# Autodesk Inventor assembly: Montagem para cotas
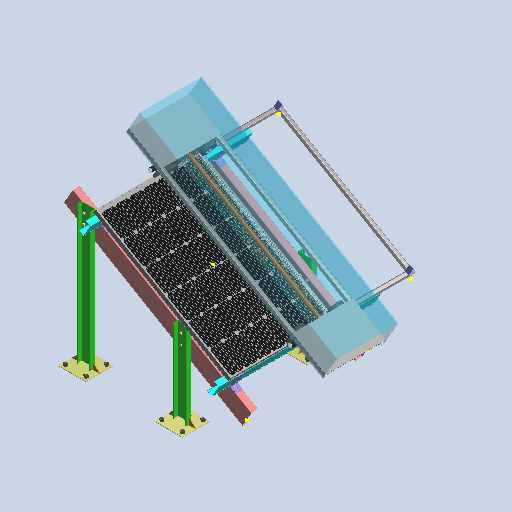
[picture p0: Inventor's stored thumbnail of the model, 512x512]
Saved by Autodesk Inventor 2026.2 (Build 302298010, 298A)
## iProperties
Created: 2019-12-15
Part Number: Montagem para cotas
Document SubType Name: Assembly
Designer: Rubens
Sending System: SolidWorks 2021
Last Author: Mohsen
Last Saved: 2022-08-25
Author: Rubens
## Documents named in this file (29)
- C:\Users\Rubens\Downloads\TCC1803\TCC 1703\Projeto TCC\Main_Solar_Structure\Montagem para cotas.iam
- C:\Users\Rubens\Downloads\TCC1803\TCC 1703\Projeto TCC\Main_Solar_Structure\Small_Column.ipt
- C:\Users\Rubens\Downloads\TCC1803\TCC 1703\Projeto TCC\Main_Solar_Structure\Large_Column.ipt
- C:\Users\Rubens\Downloads\TCC1803\TCC 1703\Projeto TCC\Main_Solar_Structure\Bottom_Beam.ipt
- C:\Users\Rubens\Downloads\TCC1803\TCC 1703\Projeto TCC\Main_Solar_Structure\Base_Plate.ipt
- C:\Users\Rubens\Downloads\TCC1803\TCC 1703\Projeto TCC\Main_Solar_Structure\Base_Support.ipt
- C:\Users\Rubens\Downloads\TCC1803\TCC 1703\Projeto TCC\Main_Solar_Structure\Beam_Support.ipt
- C:\Users\Rubens\Downloads\TCC1803\TCC 1703\Projeto TCC\Main_Solar_Structure\M10_Screw&Nut.iam
- C:\Users\Rubens\Downloads\TCC1803\TCC 1703\Projeto TCC\Main_Solar_Structure\ISO - 4034 - M16 - S_.ipt
- C:\Users\Rubens\Downloads\TCC1803\TCC 1703\Projeto TCC\Main_Solar_Structure\Base_Plate_MIR.ipt
- C:\Users\Rubens\Downloads\TCC1803\TCC 1703\Projeto TCC\Main_Solar_Structure\Base_Support_MIR.ipt
- C:\Users\Rubens\Downloads\TCC1803\TCC 1703\Projeto TCC\Main_Solar_Structure\ISO - 4034 - M16 - S__MIR.ipt
- C:\Users\Rubens\Downloads\TCC1803\TCC 1703\Projeto TCC\Main_Solar_Structure\Top_Beam_2780.ipt
- C:\Users\Rubens\Downloads\TCC1803\TCC 1703\Projeto TCC\Main_Solar_Structure\Perfil tubo - 30x30x3.ipt
- C:\Users\Rubens\Downloads\TCC1803\TCC 1703\Projeto TCC\Main_Solar_Structure\tubo 30 x 30 x 3  - 500.ipt
- C:\Users\Rubens\Downloads\TCC1803\TCC 1703\Projeto TCC\Main_Solar_Structure\Limitador.ipt
- C:\Users\Rubens\Downloads\TCC1803\TCC 1703\Projeto TCC\Projeto Limpador\MontagemREVXX.iam
- C:\Users\Rubens\Downloads\TCC1803\TCC 1703\Projeto TCC\Projeto Limpador\PV ST SOLAR.ipt
- C:\Users\Rubens\Downloads\TCC1803\TCC 1703\Projeto TCC\Main_Solar_Structure\Small_Column_MIR3.ipt
- C:\Users\Rubens\Downloads\TCC1803\TCC 1703\Projeto TCC\Main_Solar_Structure\Bottom_Beam_MIR3.ipt
- C:\Users\Rubens\Downloads\TCC1803\TCC 1703\Projeto TCC\Main_Solar_Structure\Base_Plate_MIR4.ipt
- C:\Users\Rubens\Downloads\TCC1803\TCC 1703\Projeto TCC\Main_Solar_Structure\Base_Support_MIR4.ipt
- C:\Users\Rubens\Downloads\TCC1803\TCC 1703\Projeto TCC\Main_Solar_Structure\Beam_Support_MIR2.ipt
- C:\Users\Rubens\Downloads\TCC1803\TCC 1703\Projeto TCC\Main_Solar_Structure\M10_Screw&Nut_MIR2.iam
- C:\Users\Rubens\Downloads\TCC1803\TCC 1703\Projeto TCC\Main_Solar_Structure\ISO - 4034 - M16 - S__MIR2.ipt
- C:\Users\Rubens\Downloads\TCC1803\TCC 1703\Projeto TCC\Main_Solar_Structure\Base_Plate_MIR_MIR3.ipt
- C:\Users\Rubens\Downloads\TCC1803\TCC 1703\Projeto TCC\Main_Solar_Structure\Base_Support_MIR_MIR2.ipt
- C:\Users\Rubens\Downloads\TCC1803\TCC 1703\Projeto TCC\Main_Solar_Structure\ISO - 4034 - M16 - S__MIR_MIR2.ipt
- C:\Users\Rubens\Downloads\TCC1803\TCC 1703\Projeto TCC\Main_Solar_Structure\Large_Column_MIR4.ipt
## Components (69 placed, 28 different names)
1. Small_Column:1 — Flush:6, Mate:67
2. Bottom_Beam:1 — Mate:3, Mate:5, Mate:20, Mate:21, Mate:66, Mate:72, Angle:1, Mate:113, Mate:128, Flush:57
3. Base_Plate:1 — Flush:14
4. Base_Support:1
5. Base_Support:2
6. Base_Support:3
7. Beam_Support:3 — Mate:3, Mate:5, Mate:23
8. M10_Screw&Nut:2 [sub-assembly]
9. M10_Screw&Nut:7 [sub-assembly]
10. M10_Screw&Nut:8 [sub-assembly]
11. M10_Screw&Nut:9 [sub-assembly]
12. M10_Screw&Nut:90 [sub-assembly]
13. M10_Screw&Nut:91 [sub-assembly]
14. ISO - 4034 - M16 - S_:43
15. ISO - 4034 - M16 - S_:47
16. ISO - 4034 - M16 - S_:51
17. ISO - 4034 - M16 - S_:55
18. Base_Plate_MIR:1 — Flush:14, Mate:65
19. Base_Support_MIR:1
20. Base_Support_MIR:2
21. Base_Support_MIR:3
22. ISO - 4034 - M16 - S__MIR:1
23. ISO - 4034 - M16 - S__MIR:2
24. ISO - 4034 - M16 - S__MIR:3
25. Top_Beam_2780:1 — Mate:21, Flush:7, Flush:45, Mate:112, Mate:129, Flush:59
26. Top_Beam_2780:2 — Mate:20, Mate:23, Flush:7, Mate:107
27. ISO - 4034 - M16 - S__MIR:4 — Mate:65
28. Large_Column:1 — Mate:66, Mate:67, Mate:86, Mate:87, Mate:88, Mate:89
29. Limitador:1 — Flush:53, Flush:54, Mate:116
30. Limitador:4 — Flush:51, Flush:52, Mate:115
31. M10_Screw&Nut:92 [sub-assembly] — Mate:86
32. M10_Screw&Nut:93 [sub-assembly] — Mate:88
33. M10_Screw&Nut:94 [sub-assembly] — Mate:89
34. M10_Screw&Nut:96 [sub-assembly] — Mate:87
35. Perfil tubo - 30x30x3:3 — Flush:35, Flush:36, Mate:104, Mate:106, Flush:39, Flush:40, Mate:109
36. tubo 30 x 30 x 3  - 500:4 — Flush:35, Flush:36, Mate:104, Mate:105, Flush:37, Flush:38, Flush:43, Flush:44
37. Perfil tubo - 30x30x3:4 — Mate:105, Flush:37, Flush:38, Flush:41, Flush:51, Flush:52, Mate:115, Flush:53, Flush:54, Mate:116
38. tubo 30 x 30 x 3  - 500:5 — Mate:106, Flush:39, Flush:40, Flush:41
39. PV ST SOLAR:1 — Mate:107, Mate:109, Flush:43, Flush:44, Flush:45, Tangent:1, Tangent:2, Tangent:3, Tangent:4
40. Beam_Support:4 — Mate:112, Mate:113, Mate:128, Flush:57
41. Small_Column_MIR3:1 — Flush:55, Mate:121
42. Bottom_Beam_MIR3:1 — Mate:118, Mate:119, Mate:122, Angle:2, Mate:123, Mate:127, Flush:58, Flush:59
43. Base_Plate_MIR4:1 — Flush:56
44. Base_Support_MIR4:1
45. Base_Support_MIR4:2
46. Base_Support_MIR4:3
47. Beam_Support_MIR2:1 — Mate:118, Mate:119
48. M10_Screw&Nut_MIR2:1 [sub-assembly]
49. M10_Screw&Nut_MIR2:2 [sub-assembly]
50. M10_Screw&Nut_MIR2:3 [sub-assembly]
51. M10_Screw&Nut_MIR2:4 [sub-assembly]
52. ISO - 4034 - M16 - S__MIR2:1
53. ISO - 4034 - M16 - S__MIR2:2
54. ISO - 4034 - M16 - S__MIR2:3
55. ISO - 4034 - M16 - S__MIR2:4
56. Base_Plate_MIR_MIR3:1 — Flush:56, Mate:120
57. Base_Support_MIR_MIR2:1
58. Base_Support_MIR_MIR2:2
59. Base_Support_MIR_MIR2:3
60. ISO - 4034 - M16 - S__MIR_MIR2:1
61. ISO - 4034 - M16 - S__MIR_MIR2:2
62. ISO - 4034 - M16 - S__MIR_MIR2:3
63. ISO - 4034 - M16 - S__MIR_MIR2:4 — Mate:120
64. Large_Column_MIR4:1 — Mate:121, Mate:122, Mate:124, Mate:125, Mate:126
65. M10_Screw&Nut_MIR2:5 [sub-assembly] — Mate:124
66. M10_Screw&Nut_MIR2:6 [sub-assembly] — Mate:125
67. M10_Screw&Nut_MIR2:7 [sub-assembly] — Mate:126
68. Beam_Support_MIR2:2 — Mate:127, Mate:129, Flush:58
69. MontagemREVXX:1 [sub-assembly] — Tangent:1, Tangent:2, Tangent:3, Tangent:4
## Relationships (63: Mate 34, Flush 23, Tangent 4, Angle 2)
- Mate:3: Bottom_Beam:1 ↔ Beam_Support:3
- Mate:5: Bottom_Beam:1 ↔ Beam_Support:3
- Flush:6 (300 mm): Small_Column:1
- Mate:20: Bottom_Beam:1 ↔ Top_Beam_2780:2
- Mate:21: Bottom_Beam:1 ↔ Top_Beam_2780:1
- Mate:23: Beam_Support:3 ↔ Top_Beam_2780:2
- Flush:7: Top_Beam_2780:1 ↔ Top_Beam_2780:2
- Flush:14: Base_Plate:1 ↔ Base_Plate_MIR:1
- Mate:65: Base_Plate_MIR:1 ↔ ISO - 4034 - M16 - S__MIR:4
- Mate:66: Bottom_Beam:1 ↔ Large_Column:1
- Mate:67 (600 mm): Small_Column:1 ↔ Large_Column:1
- Mate:72: Bottom_Beam:1
- Angle:1 (0 deg): Bottom_Beam:1
- Flush:16 (-450 mm)
- Mate:86: Large_Column:1 ↔ M10_Screw&Nut:92
- Mate:87: Large_Column:1 ↔ M10_Screw&Nut:96
- Mate:88: Large_Column:1 ↔ M10_Screw&Nut:93
- Mate:89: Large_Column:1 ↔ M10_Screw&Nut:94
- Flush:35: Perfil tubo - 30x30x3:3 ↔ tubo 30 x 30 x 3  - 500:4
- Flush:36: Perfil tubo - 30x30x3:3 ↔ tubo 30 x 30 x 3  - 500:4
- Mate:104: Perfil tubo - 30x30x3:3 ↔ tubo 30 x 30 x 3  - 500:4
- Mate:105: tubo 30 x 30 x 3  - 500:4 ↔ Perfil tubo - 30x30x3:4
- Flush:37: tubo 30 x 30 x 3  - 500:4 ↔ Perfil tubo - 30x30x3:4
- Flush:38: tubo 30 x 30 x 3  - 500:4 ↔ Perfil tubo - 30x30x3:4
- Mate:106: Perfil tubo - 30x30x3:3 ↔ tubo 30 x 30 x 3  - 500:5
- Flush:39: Perfil tubo - 30x30x3:3 ↔ tubo 30 x 30 x 3  - 500:5
- Flush:40: Perfil tubo - 30x30x3:3 ↔ tubo 30 x 30 x 3  - 500:5
- Flush:41: Perfil tubo - 30x30x3:4 ↔ tubo 30 x 30 x 3  - 500:5
- Mate:107: Top_Beam_2780:2 ↔ PV ST SOLAR:1
- Mate:109: Perfil tubo - 30x30x3:3 ↔ PV ST SOLAR:1
- Flush:43: tubo 30 x 30 x 3  - 500:4 ↔ PV ST SOLAR:1
- Flush:44: tubo 30 x 30 x 3  - 500:4 ↔ PV ST SOLAR:1
- Flush:45: Top_Beam_2780:1 ↔ PV ST SOLAR:1
- Mate:112: Top_Beam_2780:1 ↔ Beam_Support:4
- Mate:113: Bottom_Beam:1 ↔ Beam_Support:4
- Flush:51: Limitador:4 ↔ Perfil tubo - 30x30x3:4
- Flush:52: Limitador:4 ↔ Perfil tubo - 30x30x3:4
- Mate:115: Limitador:4 ↔ Perfil tubo - 30x30x3:4
- Flush:53: Limitador:1 ↔ Perfil tubo - 30x30x3:4
- Flush:54: Limitador:1 ↔ Perfil tubo - 30x30x3:4
- Mate:116: Limitador:1 ↔ Perfil tubo - 30x30x3:4
- Mate:118: Bottom_Beam_MIR3:1 ↔ Beam_Support_MIR2:1
- Mate:119: Bottom_Beam_MIR3:1 ↔ Beam_Support_MIR2:1
- Flush:55 (300 mm): Small_Column_MIR3:1
- Flush:56: Base_Plate_MIR4:1 ↔ Base_Plate_MIR_MIR3:1
- Mate:120: Base_Plate_MIR_MIR3:1 ↔ ISO - 4034 - M16 - S__MIR_MIR2:4
- Mate:121 (600 mm): Small_Column_MIR3:1 ↔ Large_Column_MIR4:1
- Mate:122: Bottom_Beam_MIR3:1 ↔ Large_Column_MIR4:1
- Angle:2 (0 deg): Bottom_Beam_MIR3:1
- Mate:123: Bottom_Beam_MIR3:1
- Mate:124: Large_Column_MIR4:1 ↔ M10_Screw&Nut_MIR2:5
- Mate:125: Large_Column_MIR4:1 ↔ M10_Screw&Nut_MIR2:6
- Mate:126: Large_Column_MIR4:1 ↔ M10_Screw&Nut_MIR2:7
- Mate:127: Bottom_Beam_MIR3:1 ↔ Beam_Support_MIR2:2
- Mate:128: Bottom_Beam:1 ↔ Beam_Support:4
- Flush:57: Bottom_Beam:1 ↔ Beam_Support:4
- Mate:129: Top_Beam_2780:1 ↔ Beam_Support_MIR2:2
- Flush:58: Bottom_Beam_MIR3:1 ↔ Beam_Support_MIR2:2
- Flush:59 (180 mm): Top_Beam_2780:1 ↔ Bottom_Beam_MIR3:1
- Tangent:1: PV ST SOLAR:1 ↔ MontagemREVXX:1
- Tangent:2: PV ST SOLAR:1 ↔ MontagemREVXX:1
- Tangent:3: PV ST SOLAR:1 ↔ MontagemREVXX:1
- Tangent:4: PV ST SOLAR:1 ↔ MontagemREVXX:1
